# Autodesk Inventor assembly: servo_leg_top_frame_with_nuts_without_arduino
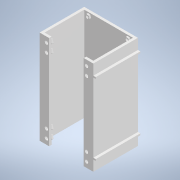
[picture p0: Inventor's stored thumbnail of the model, 180x180]
Saved by Autodesk Inventor 2021.4 (Build 254397000, 397)
## iProperties
Created: 2022-07-27
Part Number: servo_leg_top_frame_with_nuts_without_arduino
Document SubType Name: Assembly
Designer: isamu
Author: isamu
## Documents named in this file (5)
- D:\personal_projects\robot\inventor\2021_matlab_compat _v2\servo_frames\servo_leg_top_frame_with_nuts_without_arduino.iam
- D:\personal_projects\robot\exports\frames\top_of_leg_servo_frame.ipt
- D:\personal_projects\robot\exports\screws\m2 nuts.ipt
- D:\personal_projects\robot\exports\screws\m3 nuts.ipt
- D:\personal_projects\robot\exports\screws\m4 nuts.ipt
## Components (13 placed, 4 different names)
1. top_of_leg_servo_frame:1 — Insert:1, Insert:2, Insert:3, Insert:4, Insert:5, Insert:6, Insert:7, Insert:8, Insert:9, Insert:10, Insert:11, Insert:12
2. m2 nuts:1 — Insert:12
3. m2 nuts:2 — Insert:11
4. m3 nuts:1 — Insert:9
5. m3 nuts:2 — Insert:10
6. m4 nuts:1 — Insert:3
7. m4 nuts:2 — Insert:4
8. m4 nuts:3 — Insert:2
9. m4 nuts:4 — Insert:1
10. m4 nuts:5 — Insert:5
11. m4 nuts:6 — Insert:8
12. m4 nuts:7 — Insert:7
13. m4 nuts:8 — Insert:6
## Relationships (12: Insert 12)
- Insert:1: top_of_leg_servo_frame:1 ↔ m4 nuts:4
- Insert:2: top_of_leg_servo_frame:1 ↔ m4 nuts:3
- Insert:3: top_of_leg_servo_frame:1 ↔ m4 nuts:1
- Insert:4: top_of_leg_servo_frame:1 ↔ m4 nuts:2
- Insert:5: top_of_leg_servo_frame:1 ↔ m4 nuts:5
- Insert:6: top_of_leg_servo_frame:1 ↔ m4 nuts:8
- Insert:7: top_of_leg_servo_frame:1 ↔ m4 nuts:7
- Insert:8: top_of_leg_servo_frame:1 ↔ m4 nuts:6
- Insert:9: top_of_leg_servo_frame:1 ↔ m3 nuts:1
- Insert:10: top_of_leg_servo_frame:1 ↔ m3 nuts:2
- Insert:11: top_of_leg_servo_frame:1 ↔ m2 nuts:2
- Insert:12: top_of_leg_servo_frame:1 ↔ m2 nuts:1
